# Autodesk Inventor assembly: Assembly_SARS_Detector_transmisison_v0_GALAXYS8
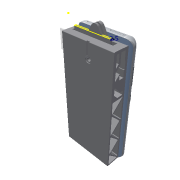
[picture p0: Inventor's stored thumbnail of the model, 180x180]
Saved by Autodesk Inventor 2019.4 (Build 234330000, 330)
## iProperties
Created: 2020-10-16
Part Number: Assembly_SARS_Detector_transmisison_v0_GALAXYS8
Document SubType Name: Assembly
Designer: diederichbenedict
Author: diederichbenedict
## Documents named in this file (5)
- C:\Users\diederichbenedict\Dropbox\Dokumente\Promotion\PROJECTS\SARSDetector\INVENTOR\SARSDetector_v0\Assembly_SARS_Detector_transmisison_v0_GALAXYS8.iam
- C:\Users\diederichbenedict\Dropbox\Dokumente\Promotion\PROJECTS\SARSDetector\INVENTOR\SARSDetector_v0\01_SARS_detector_transmission_H20P_base_v0.ipt
- C:\Users\diederichbenedict\Dropbox\Dokumente\Promotion\PROJECTS\SARSDetector\INVENTOR\SARSDetector_v0\00_LG_G3_Lens.ipt
- C:\Users\diederichbenedict\Dropbox\Dokumente\Promotion\PROJECTS\SARSDetector\INVENTOR\SARSDetector_v0\00_Microscopeslide_ZAF.ipt
- C:\Users\diederichbenedict\Dropbox\Dokumente\Promotion\PROJECTS\SARSDetector\INVENTOR\SARSDetector_v0\S8.ipt
## Components (5 placed, 4 different names)
1. 01_SARS_detector_transmission_H20P_base_v0:1 — Mate:2, Angle:1, Flush:1
2. 00_LG_G3_Lens:1 — Insert:2
3. 00_Microscopeslide_ZAF:1 — Insert:2, Angle:2
4. S8:1 — Mate:2, Angle:1, Flush:1, Insert:3, Angle:2
5. 00_LG_G3_Lens:2 — Insert:3
## Relationships (6: Insert 2, Angle 2, Mate 1, Flush 1)
- Insert:2 (0.5 mm): 00_LG_G3_Lens:1 ↔ 00_Microscopeslide_ZAF:1
- Mate:2: 01_SARS_detector_transmission_H20P_base_v0:1 ↔ S8:1
- Angle:1 (180 deg): 01_SARS_detector_transmission_H20P_base_v0:1 ↔ S8:1
- Flush:1: 01_SARS_detector_transmission_H20P_base_v0:1 ↔ S8:1
- Insert:3 (1 mm): S8:1 ↔ 00_LG_G3_Lens:2
- Angle:2 (0 deg): 00_Microscopeslide_ZAF:1 ↔ S8:1
